# Autodesk Inventor assembly: MIR_HbSocketU02ForChild
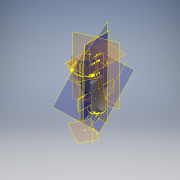
[picture p0: Inventor's stored thumbnail of the model, 180x180]
Saved by Autodesk Inventor 2017 (Build 210142000, 142)
## iProperties
Created: 2015-02-09
Part Number: MIR_HbSocketU02ForChild
Document SubType Name: Assembly
Designer: sktom
Author: Yamaura
## Documents named in this file (11)
- D:\OneDrive\CAD\MAJ\hackberry\HACKberry-hardware\3D_69%inlength\Inventor\HbSocketU02ForChild\MIR_HbSocketU02ForChild.iam
- D:\OneDrive\CAD\MAJ\hackberry\HACKberry-hardware\3D_69%inlength\Inventor\HbSocketU02ForChild\MIR_HbBatteryHingeC03.ipt
- D:\OneDrive\CAD\MAJ\hackberry\HACKberry-hardware\3D_69%inlength\Inventor\HbSocketU02ForChild\MIR_HbBatteryHingeB03.ipt
- D:\OneDrive\CAD\MAJ\hackberry\HACKberry-hardware\3D_69%inlength\Inventor\HbSocketU02ForChild\MIR_HbBatteryHingeA03.ipt
- D:\OneDrive\CAD\MAJ\hackberry\HACKberry-hardware\3D_69%inlength\Inventor\HbSocketU02ForChild\MIR_HbBatteryDoor03.ipt
- D:\OneDrive\CAD\MAJ\hackberry\HACKberry-hardware\3D_69%inlength\Inventor\HbSocketU02ForChild\MIR_HbMainFrameA01.ipt
- D:\OneDrive\CAD\MAJ\hackberry\HACKberry-hardware\3D_69%inlength\Inventor\HbSocketU02ForChild\MIR_HbBatteryDoorKnob03.ipt
- D:\OneDrive\CAD\MAJ\hackberry\HACKberry-hardware\3D_69%inlength\Inventor\HbSocketU02ForChild\MIR_HbMainFrameB01.ipt
- D:\OneDrive\CAD\MAJ\hackberry\HACKberry-hardware\3D_69%inlength\Inventor\HbSocketU02ForChild\MIR_HbBatteryDoorLever03.ipt
- D:\OneDrive\CAD\MAJ\hackberry\HACKberry-hardware\3D_69%inlength\Inventor\HbBatteryS\MIR_CR123A.ipt
- D:\OneDrive\CAD\MAJ\hackberry\HACKberry-hardware\3D_69%inlength\Inventor\HbSocketU02ForChild\HbCircuit\MIR_S7V7F5.ipt
## Components (12 placed, 10 different names)
1. MIR_HbBatteryHingeC03:1 — 挿入:7, 挿入:6
2. MIR_HbBatteryHingeB03:1 — 挿入:9, 挿入:8
3. MIR_HbBatteryHingeA03:1 — 挿入:11, 挿入:10
4. MIR_HbBatteryDoor03:1 — 挿入:11, 挿入:10, 挿入:9, 挿入:8, 挿入:7, 挿入:6, 挿入:12
5. MIR_HbMainFrameA01:1 — 挿入:5, 挿入:4, メイト:2, メイト:1, メイト:3
6. MIR_HbBatteryDoorKnob03:1 — メイト:2, メイト:1, 挿入:3
7. MIR_HbMainFrameB01:1 — 挿入:12, 挿入:5, 挿入:4, 挿入:14, 挿入:13
8. MIR_CR123A:1 — 挿入:14
9. MIR_CR123A:2 — 挿入:13
10. MIR_S7V7F5:1 — メイト:3
11. MIR_HbBatteryDoorLever03:1
12. MIR_HbBatteryDoorLever03:2 — 挿入:3
## Component patterns: (2 elements, first: MIR_HbBatteryDoorLever03:1)
## Relationships (15: Insert 12, Mate 3)
- 挿入:11 [Insert]: MIR_HbBatteryHingeA03:1 ↔ MIR_HbBatteryDoor03:1
- 挿入:10 [Insert]: MIR_HbBatteryHingeA03:1 ↔ MIR_HbBatteryDoor03:1
- 挿入:9 [Insert]: MIR_HbBatteryHingeB03:1 ↔ MIR_HbBatteryDoor03:1
- 挿入:8 [Insert]: MIR_HbBatteryHingeB03:1 ↔ MIR_HbBatteryDoor03:1
- 挿入:7 [Insert]: MIR_HbBatteryHingeC03:1 ↔ MIR_HbBatteryDoor03:1
- 挿入:6 [Insert]: MIR_HbBatteryHingeC03:1 ↔ MIR_HbBatteryDoor03:1
- 挿入:12 [Insert]: MIR_HbBatteryDoor03:1 ↔ MIR_HbMainFrameB01:1
- 挿入:5 [Insert]: MIR_HbMainFrameA01:1 ↔ MIR_HbMainFrameB01:1
- 挿入:4 [Insert]: MIR_HbMainFrameA01:1 ↔ MIR_HbMainFrameB01:1
- メイト:2 [Mate]: MIR_HbMainFrameA01:1 ↔ MIR_HbBatteryDoorKnob03:1
- メイト:1 [Mate]: MIR_HbMainFrameA01:1 ↔ MIR_HbBatteryDoorKnob03:1
- 挿入:14 [Insert]: MIR_HbMainFrameB01:1 ↔ MIR_CR123A:1
- 挿入:13 [Insert]: MIR_HbMainFrameB01:1 ↔ MIR_CR123A:2
- メイト:3 [Mate] (3 mm): MIR_HbMainFrameA01:1 ↔ MIR_S7V7F5:1
- 挿入:3 [Insert]: MIR_HbBatteryDoorKnob03:1 ↔ MIR_HbBatteryDoorLever03:2
